# Autodesk Inventor assembly: z_assembly
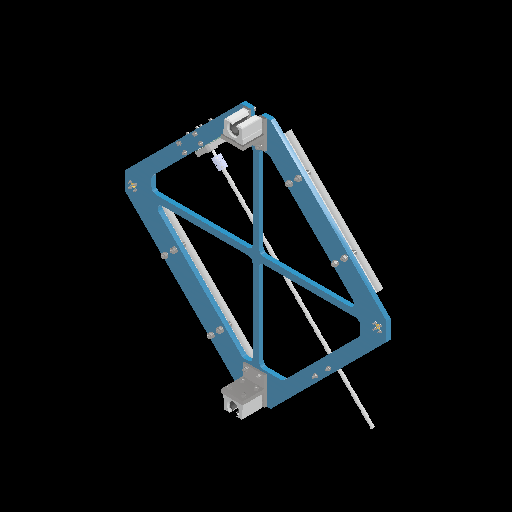
[picture p0: Inventor's stored thumbnail of the model, 512x512]
Saved by Autodesk Inventor 2026.1 (Build 301233000, 233)
## iProperties
Created: 2025-09-21
Part Number: z_assembly
Document SubType Name: Assembly
Designer: drago
Author: drago
## Documents named in this file (28)
- C:\Users\drago\Desktop\_QIST4500_Multidisciplinary_Team_Project\Proteox MX magnet positioner CAD\magnet_positioner_cad_design\z_assembly\z_assembly.iam
- C:\Users\drago\Desktop\_QIST4500_Multidisciplinary_Team_Project\Proteox MX magnet positioner CAD\magnet_positioner_cad_design\z_assembly\z_plate.ipt
- C:\Users\drago\Desktop\_QIST4500_Multidisciplinary_Team_Project\Proteox MX magnet positioner CAD\magnet_positioner_cad_design\z_assembly\y_bearing_bracket.ipt
- C:\Users\drago\Desktop\_QIST4500_Multidisciplinary_Team_Project\Proteox MX magnet positioner CAD\magnet_positioner_cad_design\z_assembly\z_bracket.ipt
- C:\Users\drago\Desktop\_QIST4500_Multidisciplinary_Team_Project\Proteox MX magnet positioner CAD\magnet_positioner_cad_design\z_assembly\y_rail.ipt
- C:\Users\drago\Desktop\_QIST4500_Multidisciplinary_Team_Project\Proteox MX magnet positioner CAD\magnet_positioner_cad_design\z_assembly\y_motor_bracket.ipt
- C:\Users\drago\Desktop\_QIST4500_Multidisciplinary_Team_Project\Proteox MX magnet positioner CAD\magnet_positioner_cad_design\other_parts\KP08.iam
- C:\Users\drago\Desktop\_QIST4500_Multidisciplinary_Team_Project\Proteox MX magnet positioner CAD\magnet_positioner_cad_design\other_parts\SBR16UU.ipt
- C:\Users\drago\Desktop\_QIST4500_Multidisciplinary_Team_Project\Proteox MX magnet positioner CAD\magnet_positioner_cad_design\other_parts\Trapezoidal lead screw Nut tr8x8-4.ipt
- C:\Users\drago\Desktop\_QIST4500_Multidisciplinary_Team_Project\Proteox MX magnet positioner CAD\magnet_positioner_cad_design\other_parts\Stepping_Motor_Nema17_34mm.ipt
- C:\Users\drago\Desktop\_QIST4500_Multidisciplinary_Team_Project\Proteox MX magnet positioner CAD\magnet_positioner_cad_design\other_parts\5X8_COUPLER.ipt
- C:\Users\drago\Desktop\_QIST4500_Multidisciplinary_Team_Project\Proteox MX magnet positioner CAD\magnet_positioner_cad_design\other_parts\Lead Screw 8mm-2.0 x 500mm.ipt
- C:\Users\drago\Documents\Inventor\Content Center Files\R2026\en-US\ISO 7089\ISO 7089 - 4 - 140 HV(1).ipt
- C:\Users\drago\Documents\Inventor\Content Center Files\R2026\en-US\ISO 4762(2)\ISO 4762 - M4 x 30ISO.ipt
- C:\Users\drago\Documents\Inventor\Content Center Files\R2026\en-US\ISO 4032(2)\ISO 4032 - M4 - ISO.ipt
- C:\Users\drago\Documents\Inventor\Content Center Files\R2026\en-US\ISO 4762(2)\ISO 4762 - M4 x 20ISO.ipt
- C:\Users\drago\Documents\Inventor\Content Center Files\R2026\en-US\ISO 7089\ISO 7089 - 6 - 140 HV(1).ipt
- C:\Users\drago\Documents\Inventor\Content Center Files\R2026\en-US\ISO 4032(2)\ISO 4032 - M6 - ISO.ipt
- C:\Users\drago\Documents\Inventor\Content Center Files\R2026\en-US\ISO 4762(2)\ISO 4762 - M6 x 25ISO.ipt
- C:\Users\drago\Documents\Inventor\Content Center Files\R2026\en-US\ISO 4762(2)\ISO 4762 - M5 x 16ISO.ipt
- C:\Users\drago\Documents\Inventor\Content Center Files\R2026\en-US\ISO 7089\ISO 7089 - 5 - 140 HV(1).ipt
- C:\Users\drago\Documents\Inventor\Content Center Files\R2026\en-US\ISO 4032(2)\ISO 4032 - M5 - ISO.ipt
- C:\Users\drago\Documents\Inventor\Content Center Files\R2026\en-US\ISO 4762(2)\ISO 4762 - M5 x 25ISO.ipt
- C:\Users\drago\Documents\Inventor\Content Center Files\R2026\en-US\ISO 4762(2)\ISO 4762 - M3 x 20ISO.ipt
- C:\Users\drago\Documents\Inventor\Content Center Files\R2026\en-US\ISO 4032(2)\ISO 4032 - M3 - ISO.ipt
- C:\Users\drago\Documents\Inventor\Content Center Files\R2026\en-US\ISO 7089\ISO 7089 - 3 - 140 HV(1).ipt
- C:\Users\drago\Documents\Inventor\Content Center Files\R2026\en-US\ISO 4762(2)\ISO 4762 - M3 x 30ISO.ipt
- C:\Users\drago\Documents\Inventor\Content Center Files\R2026\en-US\ISO 4762(2)\ISO 4762 - M3 x 10ISO.ipt
## Components (119 placed, 27 different names)
1. z_plate:1 — Mate:41, Mate:42, Mate:65, Mate:69, Mate:70, Mate:71, Mate:72, Mate:73, Mate:74, Mate:75, Mate:76, Mate:77, Mate:78, Mate:79, Mate:80, Mate:81, Mate:95, Mate:96, Mate:97, Mate:98, Mate:99, Mate:100, Mate:107, Mate:108, Mate:109, Mate:110, Mate:112, Mate:113, Mate:114, Mate:116, Mate:117, Mate:118, Mate:119, Mate:120, Mate:121, Mate:122, Mate:123, Mate:124, Mate:125, Mate:134, Mate:136, Mate:137, Mate:138, Mate:140, Mate:141, Mate:142, Mate:144, Mate:145, Mate:146, Mate:148, Mate:149, Mate:150, Mate:152, Mate:153, Mate:154, Mate:156, Mate:157, Mate:158, Mate:160, Mate:161, Mate:162, Mate:164, Mate:165, Mate:194, Mate:195, Mate:196, Mate:197, Mate:206, Mate:207, Mate:208, Mate:209, Mate:210, Mate:211, Mate:212, Mate:214, Mate:215, Mate:216, Mate:218, Mate:219, Mate:220, Mate:222, Mate:223, Mate:224, Mate:226, Mate:228, Mate:229, Mate:230, Mate:232, Mate:233, Mate:234, Mate:236, Mate:237, Mate:238, Mate:240, Mate:241, Mate:242, Mate:244, Mate:245, Mate:246, Mate:248, Mate:249, Mate:250, Mate:252, Mate:253, Mate:254, Mate:256, Mate:257
2. y_bearing_bracket:1 — Mate:65, Mate:84, Mate:85, Mate:86, Mate:109
3. z_bracket:1 — Mate:75, Mate:77, Mate:78, Mate:87, Mate:89, Mate:90, Mate:170, Mate:171, Mate:172, Mate:173, Mate:174, Mate:175, Mate:176, Mate:177, Mate:213, Mate:217
4. y_rail:1 — Mate:72, Mate:73, Mate:74, Mate:143, Mate:147, Mate:159, Mate:163
5. z_bracket:2 — Mate:76, Mate:79, Mate:80, Mate:88, Mate:91, Mate:92, Mate:178, Mate:179, Mate:180, Mate:181, Mate:182, Mate:183, Mate:184, Mate:185, Mate:221, Mate:225
6. y_rail:2 — Mate:69, Mate:70, Mate:71, Mate:135, Mate:139, Mate:151, Mate:155
7. y_motor_bracket:1 — Mate:81, Mate:101, Mate:102, Mate:103, Mate:107, Mate:108, Mate:258, Mate:259, Mate:260, Mate:261, Mate:262, Mate:263, Mate:264, Mate:265
8. KP08:1 [sub-assembly] — Mate:84, Mate:85, Mate:86, Mate:105, Mate:111, Mate:115
9. SBR16UU:1 — Mate:87, Mate:89, Mate:90
10. SBR16UU:2 — Mate:88, Mate:91, Mate:92
11. Trapezoidal lead screw Nut tr8x8-4:1 — Mate:95, Mate:96, Mate:97, Mate:243, Mate:247, Mate:251, Mate:255
12. Trapezoidal lead screw Nut tr8x8-4:2 — Mate:98, Mate:99, Mate:100, Mate:227, Mate:231, Mate:235, Mate:239
13. Stepping_Motor_Nema17_34mm:1 — Mate:93, Mate:94, Mate:101, Mate:102, Mate:103, Mate:106
14. 5X8_COUPLER:1 — Mate:93, Mate:94, Mate:104
15. Lead Screw 8mm-2.0 x 500mm:1 — Mate:104, Mate:105, Mate:106
16. ISO 7089 4:1 — Mate:110, Mate:111, Insert:1
17. ISO 4762 M4 x 30:1 — Insert:1
18. ISO 7089 4:2 — Mate:112, Mate:113, Insert:2
19. ISO 4032 M4:1 — Insert:2
20. ISO 7089 4:3 — Mate:114, Mate:115, Insert:3
21. ISO 4762 M4 x 30:2 — Insert:3
22. ISO 7089 4:4 — Mate:116, Mate:117, Insert:4
23. ISO 4032 M4:2 — Insert:4
24. ISO 7089 3:1 — Mate:258, Mate:259, Insert:47
25. ISO 4762 M3 x 30:1 — Insert:47
26. ISO 7089 3:2 — Mate:260, Mate:261, Insert:48
27. ISO 4762 M3 x 30:2 — Insert:48
28. ISO 7089 3:3 — Mate:262, Mate:263, Insert:49
29. ISO 4762 M3 x 10:1 — Insert:49
30. ISO 7089 3:4 — Mate:264, Mate:265, Insert:50
31. ISO 4762 M3 x 30:3 — Insert:50
32. ISO 7089 4:5 — Mate:118, Mate:119, Insert:5
33. ISO 4762 M4 x 20:1 — Insert:5
34. ISO 7089 4:6 — Mate:120, Mate:121, Insert:6
35. ISO 4762 M4 x 20:2 — Insert:6
36. ISO 7089 4:7 — Mate:122, Mate:123, Insert:7
37. ISO 4762 M4 x 20:3 — Insert:7
38. ISO 7089 4:8 — Mate:124, Mate:125, Insert:8
39. ISO 4762 M4 x 20:4 — Insert:8
40. ISO 4762 M6 x 25:1 — Mate:134, Mate:135
41. ISO 7089 6:3 — Mate:136, Mate:137, Insert:11
42. ISO 4032 M6:2 — Insert:11
43. ISO 4762 M6 x 25:2 — Mate:138, Mate:139
44. ISO 7089 6:4 — Mate:140, Mate:141, Insert:12
45. ISO 4032 M6:3 — Insert:12
46. ISO 4762 M6 x 25:3 — Mate:142, Mate:143
47. ISO 7089 6:5 — Mate:144, Mate:145, Insert:13
48. ISO 4032 M6:4 — Insert:13
49. ISO 4762 M6 x 25:4 — Mate:146, Mate:147
50. ISO 7089 6:6 — Mate:148, Mate:149, Insert:14
51. ISO 4032 M6:5 — Insert:14
52. ISO 4762 M6 x 25:5 — Mate:150, Mate:151
53. ISO 7089 6:7 — Mate:152, Mate:153, Insert:15
54. ISO 4032 M6:6 — Insert:15
55. ISO 4762 M6 x 25:6 — Mate:154, Mate:155
56. ISO 7089 6:8 — Mate:156, Mate:157, Insert:16
57. ISO 4032 M6:7 — Insert:16
58. ISO 4762 M6 x 25:7 — Mate:158, Mate:159
59. ISO 7089 6:9 — Mate:160, Mate:161, Insert:17
60. ISO 4032 M6:8 — Insert:17
61. ISO 4762 M6 x 25:8 — Mate:162, Mate:163
62. ISO 7089 6:10 — Mate:164, Mate:165, Insert:18
63. ISO 4032 M6:9 — Insert:18
64. ISO 4762 M5 x 16:1 — Insert:19
65. ISO 7089 5:1 — Mate:170, Mate:171, Insert:19
66. ISO 4762 M5 x 16:2 — Insert:20
67. ISO 7089 5:2 — Mate:172, Mate:173, Insert:20
68. ISO 7089 5:3 — Mate:174, Mate:175, Insert:21
69. ISO 4762 M5 x 16:3 — Insert:21
70. ISO 7089 5:4 — Mate:176, Mate:177, Insert:22
71. ISO 4762 M5 x 16:4 — Insert:22
72. ISO 7089 5:5 — Mate:178, Mate:179, Insert:23
73. ISO 4762 M5 x 16:5 — Insert:23
74. ISO 7089 5:6 — Mate:180, Mate:181, Insert:24
75. ISO 4762 M5 x 16:6 — Insert:24
76. ISO 7089 5:7 — Mate:182, Mate:183, Insert:25
77. ISO 4762 M5 x 16:7 — Insert:25
78. ISO 7089 5:8 — Mate:184, Mate:185, Insert:26
79. ISO 4762 M5 x 16:8 — Insert:26
80. ISO 7089 5:13 — Mate:194, Mate:195, Insert:31
81. ISO 4762 M5 x 16:9 — Insert:31
82. ISO 7089 5:14 — Mate:196, Mate:197, Insert:32
83. ISO 4762 M5 x 16:10 — Insert:32
84. ISO 7089 5:19 — Mate:206, Mate:207, Insert:37
85. ISO 4762 M5 x 16:11 — Insert:37
86. ISO 7089 5:20 — Mate:208, Mate:209, Insert:38
87. ISO 4762 M5 x 16:12 — Insert:38
88. ISO 7089 5:21 — Mate:210, Mate:211, Insert:39
89. ISO 4762 M5 x 25:1 — Insert:39
90. ISO 7089 5:22 — Mate:212, Mate:213, Insert:40
91. ISO 4032 M5:1 — Insert:40
92. ISO 7089 5:23 — Mate:214, Mate:215, Insert:41
93. ISO 4762 M5 x 25:2 — Insert:41
94. ISO 7089 5:24 — Mate:216, Mate:217, Insert:42
95. ISO 4032 M5:2 — Insert:42
96. ISO 7089 5:25 — Mate:218, Mate:219, Insert:43
97. ISO 4762 M5 x 25:3 — Insert:43
98. ISO 7089 5:26 — Mate:220, Mate:221, Insert:44
99. ISO 4032 M5:3 — Insert:44
100. ISO 7089 5:27 — Mate:222, Mate:223, Insert:45
101. ISO 4762 M5 x 25:4 — Insert:45
102. ISO 7089 5:28 — Mate:224, Mate:225, Insert:46
103. ISO 4032 M5:4 — Insert:46
104. ISO 4762 M3 x 20:1 — Mate:226, Mate:227
105. ISO 4032 M3:1 — Mate:228, Mate:229
106. ISO 4762 M3 x 20:2 — Mate:230, Mate:231
107. ISO 4032 M3:2 — Mate:232, Mate:233
108. ISO 4762 M3 x 20:3 — Mate:234, Mate:235
109. ISO 4032 M3:3 — Mate:236, Mate:237
110. ISO 4762 M3 x 20:4 — Mate:238, Mate:239
111. ISO 4032 M3:4 — Mate:240, Mate:241
112. ISO 4762 M3 x 20:5 — Mate:242, Mate:243
113. ISO 4032 M3:5 — Mate:244, Mate:245
114. ISO 4762 M3 x 20:6 — Mate:246, Mate:247
115. ISO 4032 M3:6 — Mate:248, Mate:249
116. ISO 4762 M3 x 20:7 — Mate:250, Mate:251
117. ISO 4032 M3:7 — Mate:252, Mate:253
118. ISO 4762 M3 x 20:8 — Mate:254, Mate:255
119. ISO 4032 M3:8 — Mate:256, Mate:257
## Relationships (210: Mate 170, Insert 40)
- Mate:41: z_plate:1
- Mate:42: z_plate:1
- Mate:65: z_plate:1 ↔ y_bearing_bracket:1
- Mate:69: z_plate:1 ↔ y_rail:2
- Mate:70: z_plate:1 ↔ y_rail:2
- Mate:71: z_plate:1 ↔ y_rail:2
- Mate:72: z_plate:1 ↔ y_rail:1
- Mate:73: z_plate:1 ↔ y_rail:1
- Mate:74: z_plate:1 ↔ y_rail:1
- Mate:75: z_plate:1 ↔ z_bracket:1
- Mate:76: z_plate:1 ↔ z_bracket:2
- Mate:77: z_plate:1 ↔ z_bracket:1
- Mate:78: z_plate:1 ↔ z_bracket:1
- Mate:79: z_plate:1 ↔ z_bracket:2
- Mate:80: z_plate:1 ↔ z_bracket:2
- Mate:81: z_plate:1 ↔ y_motor_bracket:1
- Mate:84: y_bearing_bracket:1 ↔ KP08:1
- Mate:85: y_bearing_bracket:1 ↔ KP08:1
- Mate:86: y_bearing_bracket:1 ↔ KP08:1
- Mate:87: z_bracket:1 ↔ SBR16UU:1
- Mate:88: z_bracket:2 ↔ SBR16UU:2
- Mate:89: z_bracket:1 ↔ SBR16UU:1
- Mate:90: z_bracket:1 ↔ SBR16UU:1
- Mate:91: z_bracket:2 ↔ SBR16UU:2
- Mate:92: z_bracket:2 ↔ SBR16UU:2
- Mate:93: Stepping_Motor_Nema17_34mm:1 ↔ 5X8_COUPLER:1
- Mate:94 (10 mm): Stepping_Motor_Nema17_34mm:1 ↔ 5X8_COUPLER:1
- Mate:95: z_plate:1 ↔ Trapezoidal lead screw Nut tr8x8-4:1
- Mate:96: z_plate:1 ↔ Trapezoidal lead screw Nut tr8x8-4:1
- Mate:97: z_plate:1 ↔ Trapezoidal lead screw Nut tr8x8-4:1
- Mate:98: z_plate:1 ↔ Trapezoidal lead screw Nut tr8x8-4:2
- Mate:99: z_plate:1 ↔ Trapezoidal lead screw Nut tr8x8-4:2
- Mate:100: z_plate:1 ↔ Trapezoidal lead screw Nut tr8x8-4:2
- Mate:101: y_motor_bracket:1 ↔ Stepping_Motor_Nema17_34mm:1
- Mate:102: y_motor_bracket:1 ↔ Stepping_Motor_Nema17_34mm:1
- Mate:103: y_motor_bracket:1 ↔ Stepping_Motor_Nema17_34mm:1
- Mate:104: 5X8_COUPLER:1 ↔ Lead Screw 8mm-2.0 x 500mm:1
- Mate:105: KP08:1 ↔ Lead Screw 8mm-2.0 x 500mm:1
- Mate:106: Stepping_Motor_Nema17_34mm:1 ↔ Lead Screw 8mm-2.0 x 500mm:1
- Mate:107: z_plate:1 ↔ y_motor_bracket:1
- Mate:108: z_plate:1 ↔ y_motor_bracket:1
- Mate:109: z_plate:1 ↔ y_bearing_bracket:1
- Mate:110: z_plate:1 ↔ ISO 7089 4:1
- Mate:111: KP08:1 ↔ ISO 7089 4:1
- Insert:1: ISO 7089 4:1 ↔ ISO 4762 M4 x 30:1
- Mate:112: z_plate:1 ↔ ISO 7089 4:2
- Mate:113: z_plate:1 ↔ ISO 7089 4:2
- Insert:2: ISO 7089 4:2 ↔ ISO 4032 M4:1
- Mate:114: z_plate:1 ↔ ISO 7089 4:3
- Mate:115: KP08:1 ↔ ISO 7089 4:3
- Insert:3: ISO 7089 4:3 ↔ ISO 4762 M4 x 30:2
- Mate:116: z_plate:1 ↔ ISO 7089 4:4
- Mate:117: z_plate:1 ↔ ISO 7089 4:4
- Insert:4: ISO 7089 4:4 ↔ ISO 4032 M4:2
- Mate:118: z_plate:1 ↔ ISO 7089 4:5
- Mate:119: z_plate:1 ↔ ISO 7089 4:5
- Insert:5: ISO 7089 4:5 ↔ ISO 4762 M4 x 20:1
- Mate:120: z_plate:1 ↔ ISO 7089 4:6
- Mate:121: z_plate:1 ↔ ISO 7089 4:6
- Insert:6: ISO 7089 4:6 ↔ ISO 4762 M4 x 20:2
- Mate:122: z_plate:1 ↔ ISO 7089 4:7
- Mate:123: z_plate:1 ↔ ISO 7089 4:7
- Insert:7: ISO 7089 4:7 ↔ ISO 4762 M4 x 20:3
- Mate:124: z_plate:1 ↔ ISO 7089 4:8
- Mate:125: z_plate:1 ↔ ISO 7089 4:8
- Insert:8: ISO 7089 4:8 ↔ ISO 4762 M4 x 20:4
- Mate:134: z_plate:1 ↔ ISO 4762 M6 x 25:1
- Mate:135: y_rail:2 ↔ ISO 4762 M6 x 25:1
- Mate:136: z_plate:1 ↔ ISO 7089 6:3
- Mate:137: z_plate:1 ↔ ISO 7089 6:3
- Insert:11: ISO 7089 6:3 ↔ ISO 4032 M6:2
- Mate:138: z_plate:1 ↔ ISO 4762 M6 x 25:2
- Mate:139: y_rail:2 ↔ ISO 4762 M6 x 25:2
- Mate:140: z_plate:1 ↔ ISO 7089 6:4
- Mate:141: z_plate:1 ↔ ISO 7089 6:4
- Insert:12: ISO 7089 6:4 ↔ ISO 4032 M6:3
- Mate:142: z_plate:1 ↔ ISO 4762 M6 x 25:3
- Mate:143: y_rail:1 ↔ ISO 4762 M6 x 25:3
- Mate:144: z_plate:1 ↔ ISO 7089 6:5
- Mate:145: z_plate:1 ↔ ISO 7089 6:5
- Insert:13: ISO 7089 6:5 ↔ ISO 4032 M6:4
- Mate:146: z_plate:1 ↔ ISO 4762 M6 x 25:4
- Mate:147: y_rail:1 ↔ ISO 4762 M6 x 25:4
- Mate:148: z_plate:1 ↔ ISO 7089 6:6
- Mate:149: z_plate:1 ↔ ISO 7089 6:6
- Insert:14: ISO 7089 6:6 ↔ ISO 4032 M6:5
- Mate:150: z_plate:1 ↔ ISO 4762 M6 x 25:5
- Mate:151: y_rail:2 ↔ ISO 4762 M6 x 25:5
- Mate:152: z_plate:1 ↔ ISO 7089 6:7
- Mate:153: z_plate:1 ↔ ISO 7089 6:7
- Insert:15: ISO 7089 6:7 ↔ ISO 4032 M6:6
- Mate:154: z_plate:1 ↔ ISO 4762 M6 x 25:6
- Mate:155: y_rail:2 ↔ ISO 4762 M6 x 25:6
- Mate:156: z_plate:1 ↔ ISO 7089 6:8
- Mate:157: z_plate:1 ↔ ISO 7089 6:8
- Insert:16: ISO 7089 6:8 ↔ ISO 4032 M6:7
- Mate:158: z_plate:1 ↔ ISO 4762 M6 x 25:7
- Mate:159: y_rail:1 ↔ ISO 4762 M6 x 25:7
- Mate:160: z_plate:1 ↔ ISO 7089 6:9
- Mate:161: z_plate:1 ↔ ISO 7089 6:9
- Insert:17: ISO 7089 6:9 ↔ ISO 4032 M6:8
- Mate:162: z_plate:1 ↔ ISO 4762 M6 x 25:8
- Mate:163: y_rail:1 ↔ ISO 4762 M6 x 25:8
- Mate:164: z_plate:1 ↔ ISO 7089 6:10
- Mate:165: z_plate:1 ↔ ISO 7089 6:10
- Insert:18: ISO 7089 6:10 ↔ ISO 4032 M6:9
- Mate:170: z_bracket:1 ↔ ISO 7089 5:1
- Mate:171: z_bracket:1 ↔ ISO 7089 5:1
- Insert:19: ISO 4762 M5 x 16:1 ↔ ISO 7089 5:1
- Mate:172: z_bracket:1 ↔ ISO 7089 5:2
- Mate:173: z_bracket:1 ↔ ISO 7089 5:2
- Insert:20: ISO 4762 M5 x 16:2 ↔ ISO 7089 5:2
- Mate:174: z_bracket:1 ↔ ISO 7089 5:3
- Mate:175: z_bracket:1 ↔ ISO 7089 5:3
- Insert:21: ISO 7089 5:3 ↔ ISO 4762 M5 x 16:3
- Mate:176: z_bracket:1 ↔ ISO 7089 5:4
- Mate:177: z_bracket:1 ↔ ISO 7089 5:4
- Insert:22: ISO 7089 5:4 ↔ ISO 4762 M5 x 16:4
- Mate:178: z_bracket:2 ↔ ISO 7089 5:5
- Mate:179: z_bracket:2 ↔ ISO 7089 5:5
- Insert:23: ISO 7089 5:5 ↔ ISO 4762 M5 x 16:5
- Mate:180: z_bracket:2 ↔ ISO 7089 5:6
- Mate:181: z_bracket:2 ↔ ISO 7089 5:6
- Insert:24: ISO 7089 5:6 ↔ ISO 4762 M5 x 16:6
- Mate:182: z_bracket:2 ↔ ISO 7089 5:7
- Mate:183: z_bracket:2 ↔ ISO 7089 5:7
- Insert:25: ISO 7089 5:7 ↔ ISO 4762 M5 x 16:7
- Mate:184: z_bracket:2 ↔ ISO 7089 5:8
- Mate:185: z_bracket:2 ↔ ISO 7089 5:8
- Insert:26: ISO 7089 5:8 ↔ ISO 4762 M5 x 16:8
- Mate:194: z_plate:1 ↔ ISO 7089 5:13
- Mate:195: z_plate:1 ↔ ISO 7089 5:13
- Insert:31: ISO 7089 5:13 ↔ ISO 4762 M5 x 16:9
- Mate:196: z_plate:1 ↔ ISO 7089 5:14
- Mate:197: z_plate:1 ↔ ISO 7089 5:14
- Insert:32: ISO 7089 5:14 ↔ ISO 4762 M5 x 16:10
- Mate:206: z_plate:1 ↔ ISO 7089 5:19
- Mate:207: z_plate:1 ↔ ISO 7089 5:19
- Insert:37: ISO 7089 5:19 ↔ ISO 4762 M5 x 16:11
- Mate:208: z_plate:1 ↔ ISO 7089 5:20
- Mate:209: z_plate:1 ↔ ISO 7089 5:20
- Insert:38: ISO 7089 5:20 ↔ ISO 4762 M5 x 16:12
- Mate:210: z_plate:1 ↔ ISO 7089 5:21
- Mate:211: z_plate:1 ↔ ISO 7089 5:21
- Insert:39: ISO 7089 5:21 ↔ ISO 4762 M5 x 25:1
- Mate:212: z_plate:1 ↔ ISO 7089 5:22
- Mate:213: z_bracket:1 ↔ ISO 7089 5:22
- Insert:40: ISO 7089 5:22 ↔ ISO 4032 M5:1
- Mate:214: z_plate:1 ↔ ISO 7089 5:23
- Mate:215: z_plate:1 ↔ ISO 7089 5:23
- Insert:41: ISO 7089 5:23 ↔ ISO 4762 M5 x 25:2
- Mate:216: z_plate:1 ↔ ISO 7089 5:24
- Mate:217: z_bracket:1 ↔ ISO 7089 5:24
- Insert:42: ISO 7089 5:24 ↔ ISO 4032 M5:2
- Mate:218: z_plate:1 ↔ ISO 7089 5:25
- Mate:219: z_plate:1 ↔ ISO 7089 5:25
- Insert:43: ISO 7089 5:25 ↔ ISO 4762 M5 x 25:3
- Mate:220: z_plate:1 ↔ ISO 7089 5:26
- Mate:221: z_bracket:2 ↔ ISO 7089 5:26
- Insert:44: ISO 7089 5:26 ↔ ISO 4032 M5:3
- Mate:222: z_plate:1 ↔ ISO 7089 5:27
- Mate:223: z_plate:1 ↔ ISO 7089 5:27
- Insert:45: ISO 7089 5:27 ↔ ISO 4762 M5 x 25:4
- Mate:224: z_plate:1 ↔ ISO 7089 5:28
- Mate:225: z_bracket:2 ↔ ISO 7089 5:28
- Insert:46: ISO 7089 5:28 ↔ ISO 4032 M5:4
- Mate:226: z_plate:1 ↔ ISO 4762 M3 x 20:1
- Mate:227: Trapezoidal lead screw Nut tr8x8-4:2 ↔ ISO 4762 M3 x 20:1
- Mate:228: z_plate:1 ↔ ISO 4032 M3:1
- Mate:229: z_plate:1 ↔ ISO 4032 M3:1
- Mate:230: z_plate:1 ↔ ISO 4762 M3 x 20:2
- Mate:231: Trapezoidal lead screw Nut tr8x8-4:2 ↔ ISO 4762 M3 x 20:2
- Mate:232: z_plate:1 ↔ ISO 4032 M3:2
- Mate:233: z_plate:1 ↔ ISO 4032 M3:2
- Mate:234: z_plate:1 ↔ ISO 4762 M3 x 20:3
- Mate:235: Trapezoidal lead screw Nut tr8x8-4:2 ↔ ISO 4762 M3 x 20:3
- Mate:236: z_plate:1 ↔ ISO 4032 M3:3
- Mate:237: z_plate:1 ↔ ISO 4032 M3:3
- Mate:238: z_plate:1 ↔ ISO 4762 M3 x 20:4
- Mate:239: Trapezoidal lead screw Nut tr8x8-4:2 ↔ ISO 4762 M3 x 20:4
- Mate:240: z_plate:1 ↔ ISO 4032 M3:4
- Mate:241: z_plate:1 ↔ ISO 4032 M3:4
- Mate:242: z_plate:1 ↔ ISO 4762 M3 x 20:5
- Mate:243: Trapezoidal lead screw Nut tr8x8-4:1 ↔ ISO 4762 M3 x 20:5
- Mate:244: z_plate:1 ↔ ISO 4032 M3:5
- Mate:245: z_plate:1 ↔ ISO 4032 M3:5
- Mate:246: z_plate:1 ↔ ISO 4762 M3 x 20:6
- Mate:247: Trapezoidal lead screw Nut tr8x8-4:1 ↔ ISO 4762 M3 x 20:6
- Mate:248: z_plate:1 ↔ ISO 4032 M3:6
- Mate:249: z_plate:1 ↔ ISO 4032 M3:6
- Mate:250: z_plate:1 ↔ ISO 4762 M3 x 20:7
- Mate:251: Trapezoidal lead screw Nut tr8x8-4:1 ↔ ISO 4762 M3 x 20:7
- Mate:252: z_plate:1 ↔ ISO 4032 M3:7
- Mate:253: z_plate:1 ↔ ISO 4032 M3:7
- Mate:254: z_plate:1 ↔ ISO 4762 M3 x 20:8
- Mate:255: Trapezoidal lead screw Nut tr8x8-4:1 ↔ ISO 4762 M3 x 20:8
- Mate:256: z_plate:1 ↔ ISO 4032 M3:8
- Mate:257: z_plate:1 ↔ ISO 4032 M3:8
- Mate:258: y_motor_bracket:1 ↔ ISO 7089 3:1
- Mate:259: y_motor_bracket:1 ↔ ISO 7089 3:1
- Insert:47: ISO 7089 3:1 ↔ ISO 4762 M3 x 30:1
- Mate:260: y_motor_bracket:1 ↔ ISO 7089 3:2
- Mate:261: y_motor_bracket:1 ↔ ISO 7089 3:2
- Insert:48: ISO 7089 3:2 ↔ ISO 4762 M3 x 30:2
- Mate:262: y_motor_bracket:1 ↔ ISO 7089 3:3
- Mate:263: y_motor_bracket:1 ↔ ISO 7089 3:3
- Insert:49: ISO 7089 3:3 ↔ ISO 4762 M3 x 10:1
- Mate:264: y_motor_bracket:1 ↔ ISO 7089 3:4
- Mate:265: y_motor_bracket:1 ↔ ISO 7089 3:4
- Insert:50: ISO 7089 3:4 ↔ ISO 4762 M3 x 30:3
